# Autodesk Inventor assembly: Schwimmkoerper
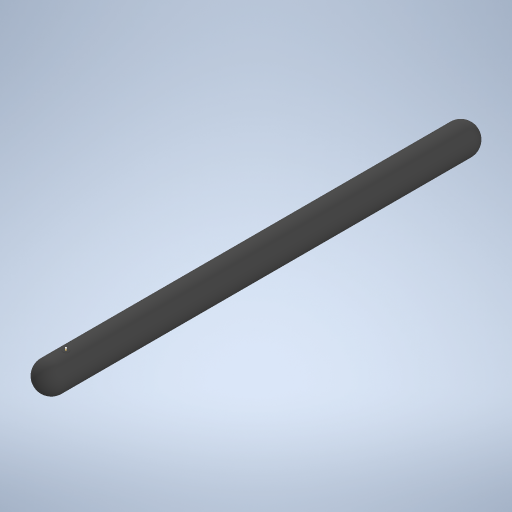
[picture p0: Inventor's stored thumbnail of the model, 512x512]
Saved by Autodesk Inventor 2024.4 (Build 284460000, 460)
## iProperties
Created: 2026-01-10
Part Number: Schwimmkoerper
Description: Schwimmkoerper
Document SubType Name: Assembly
Designer: Philf
Author: Philf
## Documents named in this file (3)
- C:\Users\Philf\Documents\Vault\Daten\I60-Konstruktion\I60-Gruppe-7\Schwimmkoerper\Schwimmkoerper.iam
- C:\Users\Philf\Documents\Vault\Daten\I60-Konstruktion\I60-Gruppe-7\Schwimmkoerper\Wulst.ipt
- C:\Users\Philf\Documents\Vault\Daten\I60-Konstruktion\I60-Gruppe-7\Schwimmkoerper\Ventil_Schrader\Schrader_plug_valve.iam
## Components (2 placed, 2 different names)
1. Wulst:1 — Passend:1, Passend:2
2. Schrader_plug_valve:1 [sub-assembly] — Passend:1, Passend:2
## Relationships (2: Mate 2)
- Passend:1 [Mate]: Wulst:1 ↔ Schrader_plug_valve:1
- Passend:2 [Mate] (-98 mm): Wulst:1 ↔ Schrader_plug_valve:1
